# Autodesk Inventor assembly: LED Assembly
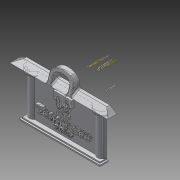
[picture p0: Inventor's stored thumbnail of the model, 180x180]
Saved by Autodesk Inventor 2018 (Build 220112000, 112)
## iProperties
Created: 2017-12-07
Part Number: LED Assembly
Document SubType Name: Assembly
Designer: Rus
Author: Rus
## Documents named in this file (3)
- E:\Libraries\Documents\3D Models\2017 TN Tech Ornament\LED Assembly.iam
- E:\Libraries\Documents\3D Models\2017 TN Tech Ornament\LED.ipt
- E:\Libraries\Documents\3D Models\2017 TN Tech Ornament\3D Printed2 LED.ipt
## Components (11 placed, 2 different names)
1. LED:1 — Angle:2, Angle:18, Insert:1
2. 3D Printed2 LED:1 — Angle:2, Angle:3, Angle:4, Angle:5, Angle:6, Angle:7, Angle:8, Angle:9, Angle:10, Angle:11, Angle:12, Angle:13, Angle:14, Angle:15, Angle:16, Angle:17, Angle:18, Insert:1
3. LED:2 — Angle:4, Angle:16
4. LED:3 — Angle:5, Angle:15
5. LED:4 — Angle:3, Angle:17
6. LED:5 — Angle:9
7. LED:6 — Angle:7, Angle:13
8. LED:7 — Angle:8, Angle:11
9. LED:8 — Angle:6, Angle:14
10. LED:9 — Angle:10
11. LED:10 — Angle:12
## Relationships (18: Angle 17, Insert 1)
- Angle:2 (0 deg): LED:1 ↔ 3D Printed2 LED:1
- Angle:3 (0 deg): 3D Printed2 LED:1 ↔ LED:4
- Angle:4 (0 deg): 3D Printed2 LED:1 ↔ LED:2
- Angle:5 (0 deg): 3D Printed2 LED:1 ↔ LED:3
- Angle:6 (0 deg): 3D Printed2 LED:1 ↔ LED:8
- Angle:7 (0 deg): 3D Printed2 LED:1 ↔ LED:6
- Angle:8 (0 deg): 3D Printed2 LED:1 ↔ LED:7
- Angle:9 (0 deg): 3D Printed2 LED:1 ↔ LED:5
- Angle:10 (0 deg): 3D Printed2 LED:1 ↔ LED:9
- Angle:11 (0 deg): 3D Printed2 LED:1 ↔ LED:7
- Angle:12 (0 deg): 3D Printed2 LED:1 ↔ LED:10
- Angle:13 (0 deg): 3D Printed2 LED:1 ↔ LED:6
- Angle:14 (0 deg): 3D Printed2 LED:1 ↔ LED:8
- Angle:15 (0 deg): 3D Printed2 LED:1 ↔ LED:3
- Angle:16 (0 deg): 3D Printed2 LED:1 ↔ LED:2
- Angle:17 (0 deg): 3D Printed2 LED:1 ↔ LED:4
- Angle:18 (0 deg): LED:1 ↔ 3D Printed2 LED:1
- Insert:1: LED:1 ↔ 3D Printed2 LED:1
